# Autodesk Inventor assembly: frame side assembly
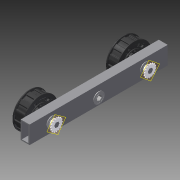
[picture p0: Inventor's stored thumbnail of the model, 180x180]
Saved by Autodesk Inventor 2015 (Build 190159000, 159)
## iProperties
Created: 2014-07-18
Part Number: frame side assembly
Document SubType Name: Assembly
Designer: Austin
Author: Austin
## Documents named in this file (6)
- C:\Users\Austin\Documents\GitHub\2014-2015\CAD\west coast drive\frame side assembly.iam
- C:\Users\Austin\Documents\GitHub\2014-2015\CAD\COTSParts\Sprockets - AndyMark\25 sprocket 16T 500Hex.ipt
- C:\Users\Austin\Documents\GitHub\2014-2015\CAD\COTSParts\Bearings - VexPro\Flanged Bearing - 0.5in Hex ID x 1.125in OD.ipt
- C:\Users\Austin\Documents\GitHub\2014-2015\CAD\west coast drive\side 1.ipt
- C:\Users\Austin\Documents\GitHub\2014-2015\CAD\west coast drive\Wheel Vexpro 4in .iam
- C:\Users\Austin\Documents\GitHub\2014-2015\CAD\west coast drive\.5 inch hex axle.ipt
## Components (13 placed, 5 different names)
1. Roller Chain Sprocket2:1 — Mate:28, Mate:29, Mate:30, Flush:9
2. Roller Chain Sprocket2:2 — Mate:35, Mate:36, Flush:12
3. Flanged Bearing - 0.5in Hex ID x 1.125in OD:1
4. Flanged Bearing - 0.5in Hex ID x 1.125in OD:2
5. side 1:1
6. Wheel Vexpro 4in :1 [sub-assembly] — Mate:31, Mate:32, Flush:10
7. Wheel Vexpro 4in :2 [sub-assembly] — Mate:37, Mate:38, Flush:13
8. Flanged Bearing - 0.5in Hex ID x 1.125in OD:3 — Mate:26, Mate:27, Flush:8
9. Flanged Bearing - 0.5in Hex ID x 1.125in OD:4
10. Flanged Bearing - 0.5in Hex ID x 1.125in OD:5
11. Flanged Bearing - 0.5in Hex ID x 1.125in OD:6 — Mate:33, Mate:34, Flush:11
12. .5 inch hex axle:1 — Mate:26, Mate:27, Flush:8, Mate:28, Mate:29, Mate:30, Flush:9, Mate:31, Mate:32, Flush:10
13. .5 inch hex axle:2 — Mate:33, Mate:34, Flush:11, Mate:35, Mate:36, Flush:12, Mate:37, Mate:38, Flush:13
## Relationships (32: Mate 25, Flush 7)
- [Mate]: Flanged Bearing - 0.5in Hex ID x 1.125in OD:2 ↔ side 1:1
- [Mate]: Flanged Bearing - 0.5in Hex ID x 1.125in OD:2 ↔ side 1:1
- [Mate]: Flanged Bearing - 0.5in Hex ID x 1.125in OD:1 ↔ side 1:1
- [Mate]: Flanged Bearing - 0.5in Hex ID x 1.125in OD:1 ↔ side 1:1
- [Flush]: Flanged Bearing - 0.5in Hex ID x 1.125in OD:1 ↔ Flanged Bearing - 0.5in Hex ID x 1.125in OD:2
- [Mate]: side 1:1 ↔ Flanged Bearing - 0.5in Hex ID x 1.125in OD:5
- [Mate]: side 1:1 ↔ Flanged Bearing - 0.5in Hex ID x 1.125in OD:5
- [Mate]: side 1:1 ↔ Flanged Bearing - 0.5in Hex ID x 1.125in OD:3
- [Mate]: side 1:1 ↔ Flanged Bearing - 0.5in Hex ID x 1.125in OD:4
- [Mate]: side 1:1 ↔ Flanged Bearing - 0.5in Hex ID x 1.125in OD:3
- [Mate]: side 1:1 ↔ Flanged Bearing - 0.5in Hex ID x 1.125in OD:6
- [Mate]: side 1:1 ↔ Flanged Bearing - 0.5in Hex ID x 1.125in OD:4
- [Mate]: side 1:1 ↔ Flanged Bearing - 0.5in Hex ID x 1.125in OD:6
- Mate:26: Flanged Bearing - 0.5in Hex ID x 1.125in OD:3 ↔ .5 inch hex axle:1
- Mate:27: Flanged Bearing - 0.5in Hex ID x 1.125in OD:3 ↔ .5 inch hex axle:1
- Flush:8 (12.7 mm): Flanged Bearing - 0.5in Hex ID x 1.125in OD:3 ↔ .5 inch hex axle:1
- Mate:28: Roller Chain Sprocket2:1 ↔ .5 inch hex axle:1
- Mate:29: Roller Chain Sprocket2:1 ↔ .5 inch hex axle:1
- Mate:30: Roller Chain Sprocket2:1 ↔ .5 inch hex axle:1
- Flush:9: Roller Chain Sprocket2:1 ↔ .5 inch hex axle:1
- Mate:31: Wheel Vexpro 4in :1 ↔ .5 inch hex axle:1
- Mate:32: Wheel Vexpro 4in :1 ↔ .5 inch hex axle:1
- Flush:10: Wheel Vexpro 4in :1 ↔ .5 inch hex axle:1
- Mate:33: Flanged Bearing - 0.5in Hex ID x 1.125in OD:6 ↔ .5 inch hex axle:2
- Mate:34: Flanged Bearing - 0.5in Hex ID x 1.125in OD:6 ↔ .5 inch hex axle:2
- Flush:11 (12.7 mm): Flanged Bearing - 0.5in Hex ID x 1.125in OD:6 ↔ .5 inch hex axle:2
- Mate:35: Roller Chain Sprocket2:2 ↔ .5 inch hex axle:2
- Mate:36: Roller Chain Sprocket2:2 ↔ .5 inch hex axle:2
- Flush:12: Roller Chain Sprocket2:2 ↔ .5 inch hex axle:2
- Mate:37: Wheel Vexpro 4in :2 ↔ .5 inch hex axle:2
- Mate:38: Wheel Vexpro 4in :2 ↔ .5 inch hex axle:2
- Flush:13: Wheel Vexpro 4in :2 ↔ .5 inch hex axle:2
## Named parameters: d4_d16 = 0 mm, d5_d17 = 0 mm, d6_d18 = 0 mm, d7_d19 = 0 mm, d8_d20 = 0 mm, d9_d21 = 0 mm, d10_d22 = 0 mm, d11_d23 = 0 mm
